# Autodesk Inventor assembly: Cadena
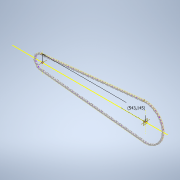
[picture p0: Inventor's stored thumbnail of the model, 180x180]
Saved by Autodesk Inventor 2021 (Build 250183000, 183)
## iProperties
Created: 2021-04-23
Part Number: Cadena
Document SubType Name: Assembly
Designer: maaro
Author: maaro
## Documents named in this file (4)
- C:\Git\Proyecto_APM\02 Inventor\bicicleta_ruta\Transmision\Cadena.iam
- C:\Git\Proyecto_APM\02 Inventor\bicicleta_ruta\Transmision\Design Accelerator\Roller Chain1.ipt
- C:\Git\Proyecto_APM\02 Inventor\bicicleta_ruta\Transmision\Eslabón 1.ipt
- C:\Git\Proyecto_APM\02 Inventor\bicicleta_ruta\Transmision\Eslabón 2.ipt
## Components (117 placed, 3 different names)
1. Roller Chain:1 — Flush:1, Flush:2, Flush:3, Mate:1, Mate:2, Angle:1
2. Eslabón 1:1 — Mate:1, Mate:2, Angle:1, Mate:5
3. Eslabón 1:2
4. Eslabón 1:3
5. Eslabón 1:4
6. Eslabón 1:5
7. Eslabón 1:6
8. Eslabón 1:7
9. Eslabón 1:8
10. Eslabón 1:9
11. Eslabón 1:10
12. Eslabón 1:11
13. Eslabón 1:12
14. Eslabón 1:13
15. Eslabón 1:14
16. Eslabón 1:15
17. Eslabón 1:16
18. Eslabón 1:17
19. Eslabón 1:18
20. Eslabón 1:19
21. Eslabón 1:20
22. Eslabón 1:21
23. Eslabón 1:22
24. Eslabón 1:23
25. Eslabón 1:24
26. Eslabón 1:25
27. Eslabón 1:26
28. Eslabón 1:27
29. Eslabón 1:28
30. Eslabón 1:29
31. Eslabón 1:30
32. Eslabón 1:31
33. Eslabón 1:32
34. Eslabón 1:33
35. Eslabón 1:34
36. Eslabón 1:35
37. Eslabón 1:36
38. Eslabón 1:37
39. Eslabón 1:38
40. Eslabón 1:39
41. Eslabón 1:40
42. Eslabón 1:41
43. Eslabón 1:42
44. Eslabón 1:43
45. Eslabón 1:44
46. Eslabón 1:45
47. Eslabón 1:46
48. Eslabón 1:47
49. Eslabón 1:48
50. Eslabón 1:49
51. Eslabón 1:50
52. Eslabón 1:51
53. Eslabón 1:52
54. Eslabón 1:53
55. Eslabón 1:54
56. Eslabón 1:55
57. Eslabón 1:56
58. Eslabón 1:57
59. Eslabón 1:58
60. Eslabón 2:1 — Mate:4, Mate:5, Angle:2
61. Eslabón 2:2
62. Eslabón 2:3
63. Eslabón 2:4
64. Eslabón 2:5
65. Eslabón 2:6
66. Eslabón 2:7
67. Eslabón 2:8
68. Eslabón 2:9
69. Eslabón 2:10
70. Eslabón 2:11
71. Eslabón 2:12
72. Eslabón 2:13
73. Eslabón 2:14
74. Eslabón 2:15
75. Eslabón 2:16
76. Eslabón 2:17
77. Eslabón 2:18
78. Eslabón 2:19
79. Eslabón 2:20
80. Eslabón 2:21
81. Eslabón 2:22
82. Eslabón 2:23
83. Eslabón 2:24
84. Eslabón 2:25
85. Eslabón 2:26
86. Eslabón 2:27
87. Eslabón 2:28
88. Eslabón 2:29
89. Eslabón 2:30
90. Eslabón 2:31
91. Eslabón 2:32
92. Eslabón 2:33
93. Eslabón 2:34
94. Eslabón 2:35
95. Eslabón 2:36
96. Eslabón 2:37
97. Eslabón 2:38
98. Eslabón 2:39
99. Eslabón 2:40
100. Eslabón 2:41
101. Eslabón 2:42
102. Eslabón 2:43
103. Eslabón 2:44
104. Eslabón 2:45
105. Eslabón 2:46
106. Eslabón 2:47
107. Eslabón 2:48
108. Eslabón 2:49
109. Eslabón 2:50
110. Eslabón 2:51
111. Eslabón 2:52
112. Eslabón 2:53
113. Eslabón 2:54
114. Eslabón 2:55
115. Eslabón 2:56
116. Eslabón 2:57
117. Eslabón 2:58
## Component patterns: (58 elements, first: Eslabón 1:1), (58 elements, first: Eslabón 2:1)
## Relationships (9: Mate 4, Flush 3, Angle 2)
- Flush:1: Roller Chain:1
- Flush:2: Roller Chain:1
- Flush:3: Roller Chain:1
- Mate:1: Roller Chain:1 ↔ Eslabón 1:1
- Mate:2: Roller Chain:1 ↔ Eslabón 1:1
- Angle:1 (0 deg): Roller Chain:1 ↔ Eslabón 1:1
- Mate:4: Eslabón 2:1
- Mate:5: Eslabón 1:1 ↔ Eslabón 2:1
- Angle:2 (180 deg): Eslabón 2:1
## Named parameters: start = 543.1451 mm
